# Autodesk Inventor assembly: CompleteSystem
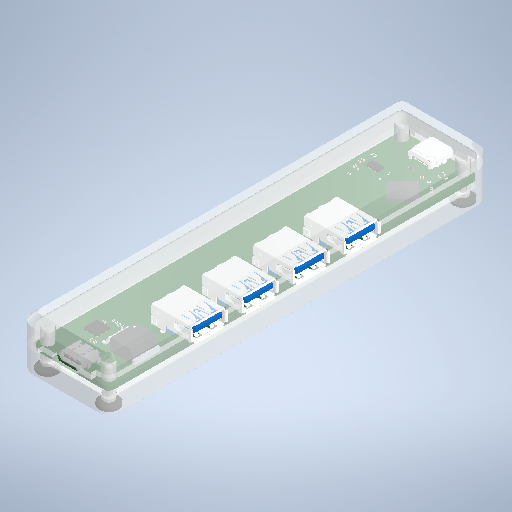
[picture p0: Inventor's stored thumbnail of the model, 512x512]
Saved by Autodesk Inventor 2025.1 (Build 291241020, 241B)
## iProperties
Created: 2026-01-18
Part Number: CompleteSystem
Document SubType Name: Assembly
Designer: JoaoVitorRamosMitidi
Author: JoaoVitorRamosMitidi
## Documents named in this file (6)
- C:\ProjectsOpenSource\USBHub3.2G1\Inventor_Project\CompleteSystem.iam
- C:\ProjectsOpenSource\USBHub3.2G1\Inventor_Project\Lower_Housing.ipt
- C:\ProjectsOpenSource\USBHub3.2G1\Inventor_Project\Board\USBHub3.2G1\USBHub3.2G1\USBHub3.2G1.ipt
- C:\ProjectsOpenSource\USBHub3.2G1\Inventor_Project\Upper_Housing.ipt
- C:\Users\JoaoVitorRamosMitidi.AzureAD\Documents\Inventor\Content Center Files\R2025\pt-BR\DIN 7985 (H)\DIN 7985 (H) - M2x10-H.ipt
- C:\ProjectsOpenSource\USBHub3.2G1\Inventor_Project\Rubber_Feet.ipt
## Components (11 placed, 5 different names)
1. Lower_Housing:1 — Coincidente:1, Inserir:1, Coincidente:2, Inserir:3, Inserir:4, Inserir:5, Inserir:6, Inserir:7, Inserir:8, Inserir:9, Inserir:10
2. USBHub3.2G1:1 — Coincidente:1, Inserir:1, Coincidente:2, Coincidente:3, Inserir:2, Coincidente:4
3. Upper_Housing:1 — Coincidente:3, Inserir:2, Coincidente:4
4. DIN 7985 (H) M2x10-H:1 — Inserir:3
5. DIN 7985 (H) M2x10-H:2 — Inserir:4
6. DIN 7985 (H) M2x10-H:3 — Inserir:5
7. DIN 7985 (H) M2x10-H:4 — Inserir:6
8. Rubber_Feet:1 — Inserir:10
9. Rubber_Feet:2 — Inserir:9
10. Rubber_Feet:3 — Inserir:8
11. Rubber_Feet:4 — Inserir:7
## Relationships (14: Insert 10, Mate 4)
- Coincidente:1 [Mate]: Lower_Housing:1 ↔ USBHub3.2G1:1
- Inserir:1: Lower_Housing:1 ↔ USBHub3.2G1:1
- Coincidente:2 [Mate]: Lower_Housing:1 ↔ USBHub3.2G1:1
- Coincidente:3 [Mate] (0.5 mm): USBHub3.2G1:1 ↔ Upper_Housing:1
- Inserir:2 (0.5 mm): USBHub3.2G1:1 ↔ Upper_Housing:1
- Coincidente:4 [Mate] (0.5 mm): USBHub3.2G1:1 ↔ Upper_Housing:1
- Inserir:3: Lower_Housing:1 ↔ DIN 7985 (H) M2x10-H:1
- Inserir:4: Lower_Housing:1 ↔ DIN 7985 (H) M2x10-H:2
- Inserir:5: Lower_Housing:1 ↔ DIN 7985 (H) M2x10-H:3
- Inserir:6: Lower_Housing:1 ↔ DIN 7985 (H) M2x10-H:4
- Inserir:7: Lower_Housing:1 ↔ Rubber_Feet:4
- Inserir:8: Lower_Housing:1 ↔ Rubber_Feet:3
- Inserir:9: Lower_Housing:1 ↔ Rubber_Feet:2
- Inserir:10: Lower_Housing:1 ↔ Rubber_Feet:1
